# Autodesk Inventor assembly: Ensamble intento 1 final
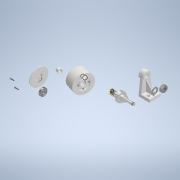
[picture p0: Inventor's stored thumbnail of the model, 180x180]
Saved by Autodesk Inventor 2021 (Build 250183000, 183)
## iProperties
Created: 2021-01-08
Part Number: Ensamble intento 1 final
Document SubType Name: Assembly
Designer: dieku
Author: dieku
## Documents named in this file (13)
- C:\Users\dieku\Documents\GitHub\tallerDibujoIngenieria\Ensambles\Ensamble intento 1 final.iam
- C:\Users\dieku\Documents\GitHub\tallerDibujoIngenieria\Partes\Eje\Eje Final.iam
- C:\Users\dieku\Documents\GitHub\tallerDibujoIngenieria\Partes\Soporte_Tensor.ipt
- C:\Users\dieku\Documents\GitHub\tallerDibujoIngenieria\Partes\anilloseparador.ipt
- C:\Users\dieku\Documents\GitHub\tallerDibujoIngenieria\Partes\Cilindro Tensor.ipt
- C:\Users\dieku\Documents\GitHub\tallerDibujoIngenieria\Partes\Tapeta Exterior.ipt
- C:\Users\dieku\Documents\GitHub\tallerDibujoIngenieria\Partes\tensorpolea.ipt
- C:\Users\dieku\Documents\Inventor\Content Center Files\R2021\en-US\DIN 934\DIN 934 - M27 x 3.ipt
- C:\Users\dieku\Documents\Inventor\Content Center Files\R2021\en-US\DIN 127 - W\DIN 127 - A 27.ipt
- C:\Users\dieku\Documents\GitHub\tallerDibujoIngenieria\Partes\Eje\Intento 1-1-2021\Ensamble 3 piezas final\DIN 912 - M6 x 1 x 16 x 13,5.ipt
- C:\Users\dieku\Documents\Inventor\Content Center Files\R2021\en-US\DIN 625 - T1\DIN 625 T1 - 6304 - 20 x 52 x 15.ipt
- C:\Users\dieku\Documents\Inventor\Content Center Files\R2021\en-US\DIN 912\DIN 912 - M6 x 1 x 25 x 22,5.ipt
- C:\Users\dieku\Documents\GitHub\tallerDibujoIngenieria\Partes\UNE 18035.ipt
## Components (16 placed, 12 different names)
1. Eje Final:1 [sub-assembly]
2. Soporte_Tensor:1
3. anilloseparador:1
4. Cilindro Tensor:1 — Mate:1, Mate:3, Mate:4
5. Tapeta Exterior:1
6. tensorpolea:1 — Mate:1, Mate:2, Mate:5
7. DIN 934 - replaced by DIN EN 24032/28673/28674 M27:1
8. DIN 127 - withdrawn A 27:1
9. DIN 912 - M6 x 1 x 16 x 13,5:1 — Mate:5
10. DIN 625 - T1 6304 - 20 x 52 x 15:1
11. DIN 912 - replaced by DIN EN ISO 4762 M6 x 25:1
12. DIN 912 - M6 x 1 x 16 x 13,5:2 — Mate:3
13. DIN 912 - M6 x 1 x 16 x 13,5:3 — Mate:2
14. DIN 912 - M6 x 1 x 16 x 13,5:4 — Mate:4
15. UNE 18035:1
16. DIN 912 - replaced by DIN EN ISO 4762 M6 x 25:2
## Relationships (5: Mate 5)
- Mate:1: Cilindro Tensor:1 ↔ tensorpolea:1
- Mate:2: tensorpolea:1 ↔ DIN 912 - M6 x 1 x 16 x 13,5:3
- Mate:3: Cilindro Tensor:1 ↔ DIN 912 - M6 x 1 x 16 x 13,5:2
- Mate:4: Cilindro Tensor:1 ↔ DIN 912 - M6 x 1 x 16 x 13,5:4
- Mate:5: tensorpolea:1 ↔ DIN 912 - M6 x 1 x 16 x 13,5:1
